# Autodesk Inventor assembly: TiltMountShort
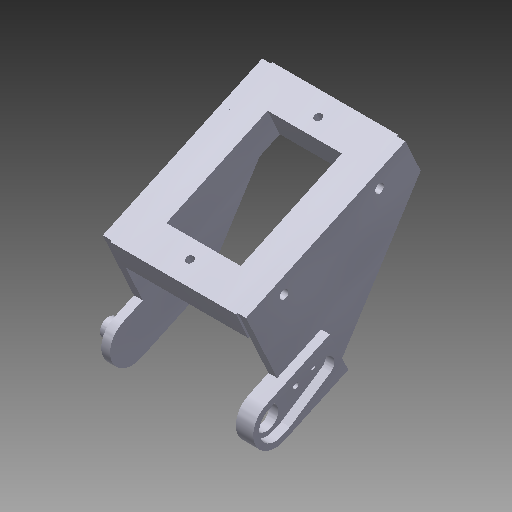
[picture p0: Inventor's stored thumbnail of the model, 512x512]
Saved by Autodesk Inventor 2017 (Build 210142000, 142)
## iProperties
Created: 2017-03-10
Part Number: TiltMountShort
Document SubType Name: Assembly
Designer: Naga
Author: Naga
## Documents named in this file (4)
- E:\GDrive\IEEE CS\SoutheastCon2017\Cad\tilt\TiltMountShort.iam
- E:\GDrive\IEEE CS\SoutheastCon2017\Cad\tilt\bottomTiltOnly.ipt
- E:\GDrive\IEEE CS\SoutheastCon2017\Cad\tilt\servoSideShort.ipt
- E:\GDrive\IEEE CS\SoutheastCon2017\Cad\tilt\sideShaftShort.ipt
## Components (3 placed, 3 different names)
1. bottomTiltOnly:1 — Mate:3, Mate:4, Mate:5, Mate:6
2. servoSideShort:1 — Mate:1, Mate:2, Mate:4, Mate:6
3. sideShaftShort:1 — Mate:1, Mate:2, Mate:3, Mate:5
## Relationships (6: Mate 6)
- Mate:1: servoSideShort:1 ↔ sideShaftShort:1
- Mate:2: servoSideShort:1 ↔ sideShaftShort:1
- Mate:3: bottomTiltOnly:1 ↔ sideShaftShort:1
- Mate:4: bottomTiltOnly:1 ↔ servoSideShort:1
- Mate:5: bottomTiltOnly:1 ↔ sideShaftShort:1
- Mate:6: bottomTiltOnly:1 ↔ servoSideShort:1
